# Autodesk Inventor assembly: OMNIWHEELV4
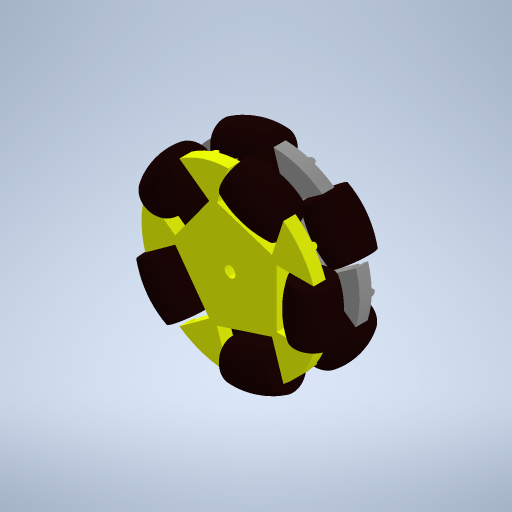
[picture p0: Inventor's stored thumbnail of the model, 512x512]
Saved by Autodesk Inventor 2024 (Build 280153000, 153)
## iProperties
Created: 2023-11-15
Part Number: OMNIWHEELV4
Document SubType Name: Assembly
Designer: felip
Author: felip
## Documents named in this file (4)
- C:\Users\felip\Downloads\Rueda Version V3\OMNIWHEELV4.iam
- C:\Users\felip\Downloads\Rueda Version V3\OmnorollerV4.ipt
- C:\Users\felip\Downloads\Rueda Version V3\Rim_H6V4.ipt
- C:\Users\felip\Downloads\Rueda Version V3\Rim_6V4.ipt
## Components (12 placed, 3 different names)
1. OmnorollerV4:1 — Rigid:3
2. Rim_H6V4:1 — Rigid:1, Rigid:2, Rigid:3, Rigid:4, Rigid:5, Rotational:1
3. OmnorollerV4:2 — Rigid:2
4. OmnorollerV4:3 — Rigid:1
5. OmnorollerV4:4 — Rigid:5
6. OmnorollerV4:5 — Rigid:4
7. Rim_6V4:1 — Rigid:6, Rigid:7, Rigid:8, Rigid:9, Rigid:10, Rotational:1
8. OmnorollerV4:6 — Rigid:9
9. OmnorollerV4:7 — Rigid:7
10. OmnorollerV4:8 — Rigid:6
11. OmnorollerV4:9 — Rigid:8
12. OmnorollerV4:10 — Rigid:10
## Relationships (11: WeldJoint 10, RevoluteJoint 1)
- Rigid:1 [WeldJoint] (4.4 mm): Rim_H6V4:1 ↔ OmnorollerV4:3
- Rigid:2 [WeldJoint] (4.4 mm): Rim_H6V4:1 ↔ OmnorollerV4:2
- Rigid:3 [WeldJoint] (4.4 mm): OmnorollerV4:1 ↔ Rim_H6V4:1
- Rigid:4 [WeldJoint] (4.4 mm): Rim_H6V4:1 ↔ OmnorollerV4:5
- Rigid:5 [WeldJoint] (4.4 mm): Rim_H6V4:1 ↔ OmnorollerV4:4
- Rigid:6 [WeldJoint] (4.4 mm): Rim_6V4:1 ↔ OmnorollerV4:8
- Rigid:7 [WeldJoint] (4.4 mm): Rim_6V4:1 ↔ OmnorollerV4:7
- Rigid:8 [WeldJoint] (4.4 mm): Rim_6V4:1 ↔ OmnorollerV4:9
- Rigid:9 [WeldJoint] (4.4 mm): Rim_6V4:1 ↔ OmnorollerV4:6
- Rigid:10 [WeldJoint] (4 mm): Rim_6V4:1 ↔ OmnorollerV4:10
- Rotational:1 [RevoluteJoint]: Rim_H6V4:1 ↔ Rim_6V4:1
